# Autodesk Inventor assembly: Wine Glass Rack Edge
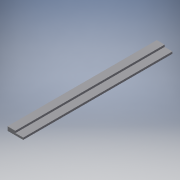
[picture p0: Inventor's stored thumbnail of the model, 180x180]
Saved by Autodesk Inventor 2016 (Build 200138000, 138)
## iProperties
Created: 2017-10-31
Part Number: Wine Glass Rack Edge
Document SubType Name: Assembly
Designer: mathaetaes
Author: mathaetaes
## Documents named in this file (3)
- C:\Users\dash.MATHAETAES\Desktop\Bar Cabinet\Wine Glass Rack Edge.iam
- C:\Users\dash.MATHAETAES\Desktop\Bar Cabinet\Wine Glass Holder Narrow.ipt
- C:\Users\dash.MATHAETAES\Desktop\Bar Cabinet\Wine Glass Holder Edge.ipt
## Components (2 placed, 2 different names)
1. Wine Glass Holder Narrow:1 — Flush:1, Mate:1, Flush:2
2. Wine Glass Holder Edge:1 — Flush:1, Mate:1, Flush:2
## Relationships (3: Flush 2, Mate 1)
- Flush:1: Wine Glass Holder Narrow:1 ↔ Wine Glass Holder Edge:1
- Mate:1: Wine Glass Holder Narrow:1 ↔ Wine Glass Holder Edge:1
- Flush:2: Wine Glass Holder Narrow:1 ↔ Wine Glass Holder Edge:1
